# Autodesk Inventor assembly: Engranajes
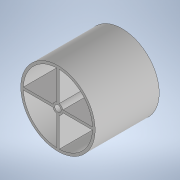
[picture p0: Inventor's stored thumbnail of the model, 180x180]
Saved by Autodesk Inventor 2021 (Build 250183000, 183)
## iProperties
Created: 2022-11-24
Part Number: Engranajes
Document SubType Name: Assembly
Designer: sergi
Author: sergi
## Documents named in this file (4)
- C:\Users\sergi\OneDrive\Escritorio\Objetos 3d\ComederoV3\Engranajes.iam
- C:\Users\sergi\OneDrive\Escritorio\Objetos 3d\ComederoV3\Engranajes\Design Accelerator\Engranajes helicoidales1.iam
- C:\Users\sergi\OneDrive\Escritorio\Objetos 3d\ComederoV3\Tambor.ipt
- C:\Users\sergi\OneDrive\Escritorio\Objetos 3d\ComederoV3\Reductora.ipt
## Components (3 placed, 3 different names)
1. Tambor:1 — Nivelación:1
2. Reductora:1 — Nivelación:1
3. Engranajes helicoidales:1 [sub-assembly]
## Relationships (1: Flush 1)
- Nivelación:1 [Flush]: Tambor:1 ↔ Reductora:1
